# Autodesk Inventor assembly: 000.500 - Второе звено
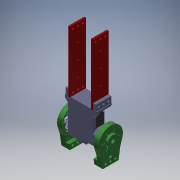
[picture p0: Inventor's stored thumbnail of the model, 180x180]
Saved by Autodesk Inventor 2019 (Build 230136000, 136)
## iProperties
Created: 2020-02-29
Part Number: 000.500 - Второе звено
Material: Типовые
Document SubType Name: Assembly
Designer: Петров Иван
Author: Петров Иван
## Documents named in this file (7)
- E:\IVAN\Ivan_desktop\GitHub\Manipulation_IRS\hardware\5-DOF\000.500 - Второе звено.iam
- E:\IVAN\Ivan_desktop\GitHub\Manipulation_IRS\hardware\5-DOF\000.501 - Держатель рычага.ipt
- E:\IVAN\Ivan_desktop\GitHub\Manipulation_IRS\hardware\5-DOF\components\Star Horn MG995.ipt
- E:\IVAN\Ivan_desktop\GitHub\Manipulation_IRS\hardware\5-DOF\components\tower prone.ipt
- E:\IVAN\Ivan_desktop\GitHub\Manipulation_IRS\hardware\5-DOF\000.502 - Стяжка.ipt
- E:\IVAN\Ivan_desktop\GitHub\Manipulation_IRS\hardware\5-DOF\components\Подшипник 626Z.ipt
- E:\IVAN\Ivan_desktop\GitHub\Manipulation_IRS\hardware\5-DOF\000.503 - Рычаг.ipt
## Components (8 placed, 6 different names)
1. 000.501 - Держатель рычага:1 — Совмещение:1, Совмещение:2, Совмещение:3
2. 000.501 - Держатель рычага:2 — Совмещение:1, Совмещение:2, Совмещение:3, Совмещение:4, Совмещение:20, Совмещение:21
3. Star Horn MG995:1 — Совмещение:4, Совмещение:7, Совмещение:8, Совмещение:20, Совмещение:21
4. tower prone:1 — Совмещение:7, Совмещение:8, Совмещение:9, Совмещение:10, Совмещение:11
5. 000.502 - Стяжка:1 — Совмещение:9, Совмещение:10, Совмещение:11, Совмещение:13, Заподлицо:1, Совмещение:14, Совмещение:15, Совмещение:16, Совмещение:17, Совмещение:18, Совмещение:19
6. Подшипник 626Z:1 — Совмещение:13, Заподлицо:1
7. 000.503 - Рычаг:1 — Совмещение:17, Совмещение:18, Совмещение:19
8. 000.503 - Рычаг:2 — Совмещение:14, Совмещение:15, Совмещение:16
## Relationships (19: Mate 18, Flush 1)
- Совмещение:1 [Mate] (40 mm): 000.501 - Держатель рычага:1 ↔ 000.501 - Держатель рычага:2
- Совмещение:2 [Mate]: 000.501 - Держатель рычага:1 ↔ 000.501 - Держатель рычага:2
- Совмещение:3 [Mate]: 000.501 - Держатель рычага:1 ↔ 000.501 - Держатель рычага:2
- Совмещение:4 [Mate]: 000.501 - Держатель рычага:2 ↔ Star Horn MG995:1
- Совмещение:7 [Mate]: Star Horn MG995:1 ↔ tower prone:1
- Совмещение:8 [Mate]: Star Horn MG995:1 ↔ tower prone:1
- Совмещение:9 [Mate]: tower prone:1 ↔ 000.502 - Стяжка:1
- Совмещение:10 [Mate]: tower prone:1 ↔ 000.502 - Стяжка:1
- Совмещение:11 [Mate]: tower prone:1 ↔ 000.502 - Стяжка:1
- Совмещение:13 [Mate]: 000.502 - Стяжка:1 ↔ Подшипник 626Z:1
- Заподлицо:1 [Flush]: 000.502 - Стяжка:1 ↔ Подшипник 626Z:1
- Совмещение:14 [Mate]: 000.502 - Стяжка:1 ↔ 000.503 - Рычаг:2
- Совмещение:15 [Mate]: 000.502 - Стяжка:1 ↔ 000.503 - Рычаг:2
- Совмещение:16 [Mate]: 000.502 - Стяжка:1 ↔ 000.503 - Рычаг:2
- Совмещение:17 [Mate]: 000.502 - Стяжка:1 ↔ 000.503 - Рычаг:1
- Совмещение:18 [Mate]: 000.502 - Стяжка:1 ↔ 000.503 - Рычаг:1
- Совмещение:19 [Mate]: 000.502 - Стяжка:1 ↔ 000.503 - Рычаг:1
- Совмещение:20 [Mate]: 000.501 - Держатель рычага:2 ↔ Star Horn MG995:1
- Совмещение:21 [Mate]: 000.501 - Держатель рычага:2 ↔ Star Horn MG995:1
